# Autodesk Inventor assembly: Assembly1
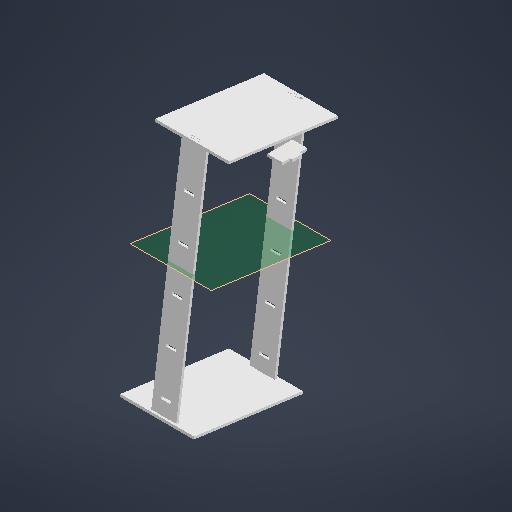
[picture p0: Inventor's stored thumbnail of the model, 512x512]
Saved by Autodesk Inventor 2026 (Build 300175050, 175E)
## iProperties
Created: 2025-06-06
Part Number: Assembly1
Document SubType Name: Assembly
Designer: HP
Author: HP
## Documents named in this file (5)
- C:\Users\HP\OneDrive\Desktop\Robotics\rack\Assembly1.iam
- C:\Users\HP\OneDrive\Desktop\Robotics\rack\Part1.ipt
- C:\Users\HP\OneDrive\Desktop\Robotics\rack\Part2.ipt
- C:\Users\HP\OneDrive\Desktop\Robotics\rack\Part3.ipt
- C:\Users\HP\OneDrive\Desktop\Robotics\rack\Part1_MIR.ipt
## Components (5 placed, 4 different names)
1. Part1:1 — Angle:1, Mate:1, Mate:2, Flush:1, Angle:3, Angle:4
2. Part2:1 — Angle:2, Mate:2, Mate:3, Mate:4
3. Part3:1
4. Part2:2 — Angle:1, Mate:1, Angle:2
5. Part1_MIR:1 — Mate:3, Mate:4, Angle:3, Angle:4
## Relationships (9: Angle 4, Mate 4, Flush 1)
- Angle:1 (90 deg): Part1:1 ↔ Part2:2
- Mate:1: Part1:1 ↔ Part2:2
- Angle:2 (0 deg): Part2:1 ↔ Part2:2
- Mate:2: Part1:1 ↔ Part2:1
- Flush:1 (-250 mm): Part1:1
- Mate:3: Part2:1 ↔ Part1_MIR:1
- Mate:4: Part2:1 ↔ Part1_MIR:1
- Angle:3 (0 deg): Part1:1 ↔ Part1_MIR:1
- Angle:4 (0 deg): Part1:1 ↔ Part1_MIR:1
